# Autodesk Inventor assembly: DynamixelXM540_no_idler_drivable
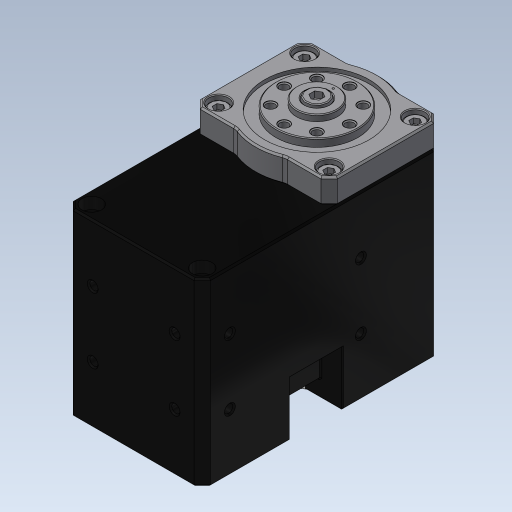
[picture p0: Inventor's stored thumbnail of the model, 512x512]
Saved by Autodesk Inventor 2023 (Build 270158000, 158)
## iProperties
Created: 2018-06-30
Part Number: DynamixelXM540_no_idler_drivable
Material: 一般
Document SubType Name: Assembly
Designer: TAKEMORI
Mass: 158.355 g
Surface Area: 205.744 cm^2
Volume: 58.65 cm^3
Density: 2.7 g/cm^3
Author: TAKEMORI
## Documents named in this file (3)
- C:\Users\michi\OneDrive - Kyoto University\lab\6_SHINOBI\FUHGA3\Design_Mechanism\Dynamixel\X540\DynamixelXM540_no_idler_toughHone.iam
- C:\Users\michi\OneDrive - Kyoto University\lab\6_SHINOBI\FUHGA3\Design_Mechanism\Dynamixel\X540\DynamixelXM540_without_hone.ipt
- C:\Users\michi\OneDrive - Kyoto University\lab\6_SHINOBI\FUHGA3\Design_Mechanism\Dynamixel\X540\EPX540-BR101.iam
## Components (2 placed, 2 different names)
1. DynamixelXM540_without_hone:1 — フラッシュ:1, フラッシュ:2, フラッシュ:3, 回転:1, 回転:2
2. EPX540-BR101:1 [sub-assembly] — 回転:1, 回転:2
## Relationships (5: Flush 3, RevoluteJoint 2)
- フラッシュ:1 [Flush]: DynamixelXM540_without_hone:1
- フラッシュ:2 [Flush]: DynamixelXM540_without_hone:1
- フラッシュ:3 [Flush]: DynamixelXM540_without_hone:1
- 回転:1 [RevoluteJoint]: DynamixelXM540_without_hone:1 ↔ EPX540-BR101:1
- 回転:2 [RevoluteJoint]: DynamixelXM540_without_hone:1 ↔ EPX540-BR101:1
